# Autodesk Inventor assembly: CNC Models
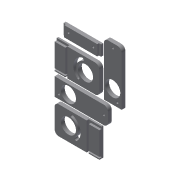
[picture p0: Inventor's stored thumbnail of the model, 180x180]
Saved by Autodesk Inventor 2018.3 (Build 223284000, 284)
## iProperties
Created: 2019-04-16
Part Number: CNC Models
Document SubType Name: Assembly
Designer: aye06091
Mass: 46.7037 g
Surface Area: 260.833 cm^2
Volume: 46.7037 cm^3
Density: 1 g/cm^3
Author: aye06091
## Documents named in this file (5)
- Y:\DeSimony-R\Senior R&D\4 R&D Shared Folder\VisiStick\VisiStick (Inventor)\Case Final\CNC Models.iam
- Y:\DeSimony-R\Senior R&D\4 R&D Shared Folder\VisiStick\VisiStick (Inventor)\Physical Parts\Lidar Sensor Case v4 Piece 2.ipt
- Y:\DeSimony-R\Senior R&D\4 R&D Shared Folder\VisiStick\VisiStick (Inventor)\Physical Parts\Lidar Sensor Case v4 Piece 1.ipt
- Y:\DeSimony-R\Senior R&D\4 R&D Shared Folder\VisiStick\VisiStick (Inventor)\Case Final\Lidar Sensor Case Piece 3.ipt
- Y:\DeSimony-R\Senior R&D\4 R&D Shared Folder\VisiStick\VisiStick (Inventor)\Physical Parts\Lidar Sensor Case v4 Piece 3.ipt
## Components (5 placed, 4 different names)
1. Lidar Sensor Case v4 Piece 2:1 — Flush:3, Flush:4, Flush:10, Flush:11, Flush:16, Mate:2
2. Lidar Sensor Case v4 Piece 1:1 — Flush:3, Flush:9
3. Lidar Sensor Case Piece 3:1 — Flush:4, Flush:9, Flush:10
4. Lidar Sensor Case v4 Piece 3:1 — Flush:11, Flush:14, Flush:15, Mate:1
5. Lidar Sensor Case v4 Piece 1:2 — Flush:14, Flush:15, Mate:1, Flush:16, Mate:2
## Relationships (10: Flush 8, Mate 2)
- Flush:3: Lidar Sensor Case v4 Piece 2:1 ↔ Lidar Sensor Case v4 Piece 1:1
- Flush:4: Lidar Sensor Case v4 Piece 2:1 ↔ Lidar Sensor Case Piece 3:1
- Flush:9: Lidar Sensor Case v4 Piece 1:1 ↔ Lidar Sensor Case Piece 3:1
- Flush:10: Lidar Sensor Case v4 Piece 2:1 ↔ Lidar Sensor Case Piece 3:1
- Flush:11: Lidar Sensor Case v4 Piece 2:1 ↔ Lidar Sensor Case v4 Piece 3:1
- Flush:14: Lidar Sensor Case v4 Piece 3:1 ↔ Lidar Sensor Case v4 Piece 1:2
- Flush:15: Lidar Sensor Case v4 Piece 3:1 ↔ Lidar Sensor Case v4 Piece 1:2
- Mate:1 (6.604 mm): Lidar Sensor Case v4 Piece 3:1 ↔ Lidar Sensor Case v4 Piece 1:2
- Flush:16: Lidar Sensor Case v4 Piece 2:1 ↔ Lidar Sensor Case v4 Piece 1:2
- Mate:2 (6.604 mm): Lidar Sensor Case v4 Piece 2:1 ↔ Lidar Sensor Case v4 Piece 1:2
